# Autodesk Inventor assembly: 오른종아리발
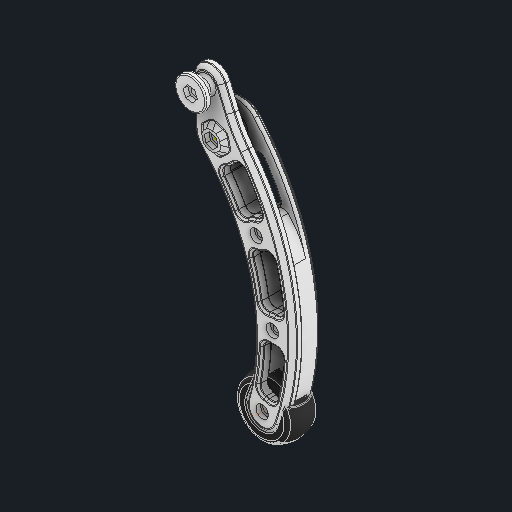
[picture p0: Inventor's stored thumbnail of the model, 512x512]
Saved by Autodesk Inventor 2027.1 (Build 311270010, 270A)
## iProperties
Created: 2026-08-22
Part Number: 오른종아리발
Document SubType Name: Assembly
Designer: moieboy9999
Mass: 19.8368 g
Surface Area: 219.095 cm^2
Volume: 30.8384 cm^3
Density: 0.643248 g/cm^3
Author: moieboy9999
## Documents named in this file (6)
- D:\micro_dog_cad\다리\프레임\오른종아리발.iam
- D:\micro_dog_cad\다리\프레임\발.ipt
- D:\micro_dog_cad\다리\프레임\축종아리베어링고정.ipt
- D:\micro_dog_cad\다리\프레임\링크 고정.ipt
- D:\micro_dog_cad\다리\프레임\종아리_MIR.ipt
- D:\micro_dog_cad\다리\프레임\링크축종아리_MIR.ipt
## Components (5 placed, 5 different names)
1. 발:1 — 메이트:5, 메이트:11, 메이트:12
2. 축종아리베어링고정:1 — 메이트:6, 메이트:7, 메이트:8, 메이트:9
3. 링크 고정:1 — 메이트:13, 메이트:14
4. 종아리_MIR:1 — 메이트:3, 메이트:4, 메이트:6, 메이트:7, 메이트:10, 메이트:11, 메이트:12
5. 링크축종아리_MIR:1 — 메이트:3, 메이트:4, 메이트:5, 메이트:8, 메이트:9, 메이트:10, 메이트:13, 메이트:14
## Relationships (12: Mate 12)
- 메이트:3 [Mate]: 종아리_MIR:1 ↔ 링크축종아리_MIR:1
- 메이트:4 [Mate]: 종아리_MIR:1 ↔ 링크축종아리_MIR:1
- 메이트:5 [Mate]: 발:1 ↔ 링크축종아리_MIR:1
- 메이트:6 [Mate]: 축종아리베어링고정:1 ↔ 종아리_MIR:1
- 메이트:7 [Mate]: 축종아리베어링고정:1 ↔ 종아리_MIR:1
- 메이트:8 [Mate]: 축종아리베어링고정:1 ↔ 링크축종아리_MIR:1
- 메이트:9 [Mate] (0.2 mm): 축종아리베어링고정:1 ↔ 링크축종아리_MIR:1
- 메이트:10 [Mate]: 종아리_MIR:1 ↔ 링크축종아리_MIR:1
- 메이트:11 [Mate]: 발:1 ↔ 종아리_MIR:1
- 메이트:12 [Mate]: 발:1 ↔ 종아리_MIR:1
- 메이트:13 [Mate]: 링크 고정:1 ↔ 링크축종아리_MIR:1
- 메이트:14 [Mate]: 링크 고정:1 ↔ 링크축종아리_MIR:1
